# Autodesk Inventor assembly: roka_asemb
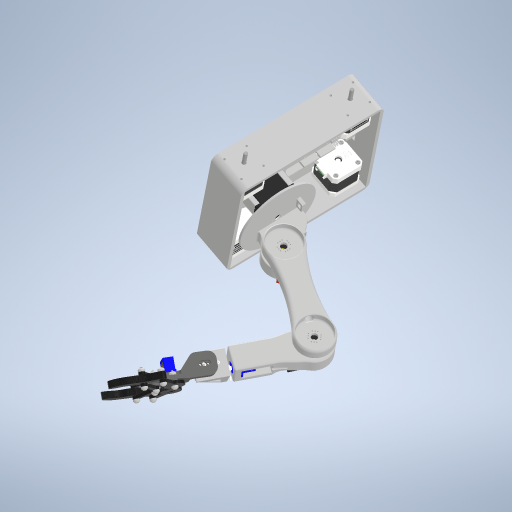
[picture p0: Inventor's stored thumbnail of the model, 512x512]
Saved by Autodesk Inventor 2024 (Build 280153000, 153)
## iProperties
Created: 2023-09-17
Part Number: roka_asemb
Document SubType Name: Assembly
Designer: jebes windows
Author: jebes windows
## Documents named in this file (19)
- C:\Users\jebes windows\Documents\Inventor\Robotska_roka\roka_asemb.iam
- C:\Users\jebes windows\Documents\Inventor\Robotska_roka\vozicek1.ipt
- C:\Users\jebes windows\Documents\Inventor\Robotska_roka\Nema 17 Motor a Pasos 17HS4401\Nema 17 Motor a Pasos 17HS4401.ipt
- C:\Users\jebes windows\Documents\Inventor\Robotska_roka\ArduinoMega_STEP_AP203\ArduinoMega_STEP_AP203.ipt
- C:\Users\jebes windows\Documents\Inventor\Robotska_roka\servo-motor-mg996r-1.snapshot.1(2)\Servo Motor MG996R  With Attachments\Servo Motor MG996R  With Attachments.iam
- C:\Users\jebes windows\Documents\Inventor\Robotska_roka\miza.ipt
- C:\Users\jebes windows\Documents\Inventor\Robotska_roka\pokrow.ipt
- C:\Users\jebes windows\Documents\Inventor\Robotska_roka\roka1.ipt
- C:\Users\jebes windows\Documents\Inventor\Robotska_roka\roka2.ipt
- C:\Users\jebes windows\Documents\Inventor\Robotska_roka\sg90-micro-servo-9g-tower-pro-1.snapshot.3\SG90 - Micro Servo 9g - Tower Pro\SG90 - Micro Servo 9g - Tower Pro.iam
- C:\Users\jebes windows\Documents\Inventor\Robotska_roka\roka3.ipt
- C:\Users\jebes windows\Documents\Inventor\Robotska_roka\Gripper_baza.ipt
- C:\Users\jebes windows\Documents\Inventor\Robotska_roka\Zobnik2.ipt
- C:\Users\jebes windows\Documents\Inventor\Robotska_roka\Zobnik1.ipt
- C:\Users\jebes windows\Documents\Inventor\Robotska_roka\povezava.ipt
- C:\Users\jebes windows\Documents\Inventor\Robotska_roka\Klesce.ipt
- C:\Users\jebes windows\Documents\Inventor\Robotska_roka\sornik1.ipt
- C:\Users\jebes windows\Documents\Inventor\Robotska_roka\matica.ipt
- C:\Users\jebes windows\Documents\Inventor\Robotska_roka\sornik_2.ipt
## Components (43 placed, 18 different names)
1. vozicek1:1 — Rigid:1, Rigid:2, Rigid:3, Rigid:4, Rigid:5, Rigid:6, Rigid:8
2. Nema 17 Motor a Pasos 17HS4401:1 — Rigid:1
3. Nema 17 Motor a Pasos 17HS4401:2 — Rigid:4
4. Nema 17 Motor a Pasos 17HS4401:3 — Rigid:3
5. Nema 17 Motor a Pasos 17HS4401:4 — Rigid:2
6. ArduinoMega_STEP_AP203:1 — Rigid:5
7. Servo Motor MG996R  With Attachments:1 [sub-assembly] — Rigid:6, Rotational:1
8. Servo Motor MG996R  With Attachments:2 [sub-assembly] — Rotational:1, Rigid:7
9. miza:1 — Rigid:7, Rigid:9
10. pokrow:1 — Rigid:8
11. Servo Motor MG996R  With Attachments:3 [sub-assembly] — Rigid:9, Rotational:2
12. Servo Motor MG996R  With Attachments:4 [sub-assembly] — Rotational:2, Rotational:3
13. roka1:1 — Rotational:3, Rotational:5
14. roka2:1 — Rigid:10, Rigid:11
15. Servo Motor MG996R  With Attachments:5 [sub-assembly] — Rigid:10
16. Servo Motor MG996R  With Attachments:6 [sub-assembly] — Rotational:5
17. SG90 - Micro Servo 9g - Tower Pro:1 [sub-assembly] — Rigid:11, Rotational:6
18. SG90 - Micro Servo 9g - Tower Pro:3 [sub-assembly] — Rigid:13, Rotational:9
19. roka3:1 — Rigid:13, Rotational:6
20. SG90 - Micro Servo 9g - Tower Pro:4 [sub-assembly] — Rigid:14, Rotational:10
21. Gripper_baza:1 — Rotational:9, Rigid:14, Rotational:11, Rotational:14, Rotational:15, Rotational:16, Rotational:17, Rotational:29
22. Zobnik2:1 — Rotational:10, Mate:1, Rotational:12, Rotation:1, Rotational:33
23. Zobnik1:1 — Rotational:11, Mate:2, Rotational:13, Rotation:1, Rotational:32, Rotational:34
24. povezava:1 — Rotational:14, Mate:3, Rotational:20, Rotational:24
25. povezava:2 — Rotational:15, Mate:4, Rotational:18, Rotational:22
26. povezava:3 — Mate:6, Rotational:17, Rotational:21, Rotational:25
27. povezava:4 — Mate:5, Rotational:16, Rotational:19, Rotational:23
28. Klesce:1 — Mate:1, Rotational:12, Mate:3, Mate:6, Rotational:31
29. Klesce:2 — Mate:2, Rotational:13, Mate:4, Mate:5, Rotational:27
30. sornik1:1 — Rotational:18
31. matica:1 — Rotational:19
32. sornik1:2 — Rotational:20
33. matica:2 — Rotational:21
34. sornik1:3 — Rotational:22
35. matica:3 — Rotational:23
36. sornik1:4 — Rotational:24
37. matica:4 — Rotational:25
38. matica:5 — Rotational:27
39. matica:6 — Rotational:29
40. matica:7 — Rotational:31
41. sornik_2:1 — Rotational:32
42. sornik_2:2 — Rotational:34
43. sornik_2:3 — Rotational:33
## Relationships (49: RevoluteJoint 29, WeldJoint 13, Mate 6, RelateRotation 1)
- Rigid:1 [WeldJoint]: vozicek1:1 ↔ Nema 17 Motor a Pasos 17HS4401:1
- Rigid:2 [WeldJoint]: vozicek1:1 ↔ Nema 17 Motor a Pasos 17HS4401:4
- Rigid:3 [WeldJoint]: vozicek1:1 ↔ Nema 17 Motor a Pasos 17HS4401:3
- Rigid:4 [WeldJoint]: vozicek1:1 ↔ Nema 17 Motor a Pasos 17HS4401:2
- Rigid:5 [WeldJoint]: vozicek1:1 ↔ ArduinoMega_STEP_AP203:1
- Rigid:6 [WeldJoint]: vozicek1:1 ↔ Servo Motor MG996R  With Attachments:1
- Rotational:1 [RevoluteJoint]: Servo Motor MG996R  With Attachments:1 ↔ Servo Motor MG996R  With Attachments:2
- Rigid:7 [WeldJoint]: Servo Motor MG996R  With Attachments:2 ↔ miza:1
- Rigid:8 [WeldJoint]: vozicek1:1 ↔ pokrow:1
- Rigid:9 [WeldJoint]: miza:1 ↔ Servo Motor MG996R  With Attachments:3
- Rotational:2 [RevoluteJoint]: Servo Motor MG996R  With Attachments:3 ↔ Servo Motor MG996R  With Attachments:4
- Rotational:3 [RevoluteJoint]: Servo Motor MG996R  With Attachments:4 ↔ roka1:1
- [RevoluteJoint]: Servo Motor MG996R  With Attachments:5 ↔ Servo Motor MG996R  With Attachments:6
- Rigid:10 [WeldJoint]: roka2:1 ↔ Servo Motor MG996R  With Attachments:5
- Rotational:5 [RevoluteJoint]: roka1:1 ↔ Servo Motor MG996R  With Attachments:6
- Rigid:11 [WeldJoint]: roka2:1 ↔ SG90 - Micro Servo 9g - Tower Pro:1
- Rigid:13 [WeldJoint]: SG90 - Micro Servo 9g - Tower Pro:3 ↔ roka3:1
- Rotational:6 [RevoluteJoint]: SG90 - Micro Servo 9g - Tower Pro:1 ↔ roka3:1
- Rotational:9 [RevoluteJoint]: SG90 - Micro Servo 9g - Tower Pro:3 ↔ Gripper_baza:1
- Rigid:14 [WeldJoint]: SG90 - Micro Servo 9g - Tower Pro:4 ↔ Gripper_baza:1
- Rotational:10 [RevoluteJoint]: SG90 - Micro Servo 9g - Tower Pro:4 ↔ Zobnik2:1
- Rotational:11 [RevoluteJoint]: Gripper_baza:1 ↔ Zobnik1:1
- Mate:1: Zobnik2:1 ↔ Klesce:1
- Rotational:12 [RevoluteJoint]: Zobnik2:1 ↔ Klesce:1
- Mate:2: Zobnik1:1 ↔ Klesce:2
- Rotational:13 [RevoluteJoint]: Zobnik1:1 ↔ Klesce:2
- Rotational:14 [RevoluteJoint]: Gripper_baza:1 ↔ povezava:1
- Mate:3: povezava:1 ↔ Klesce:1
- Rotational:15 [RevoluteJoint]: Gripper_baza:1 ↔ povezava:2
- Mate:4: povezava:2 ↔ Klesce:2
- Mate:5: povezava:4 ↔ Klesce:2
- Mate:6: povezava:3 ↔ Klesce:1
- Rotational:16 [RevoluteJoint]: Gripper_baza:1 ↔ povezava:4
- Rotational:17 [RevoluteJoint]: Gripper_baza:1 ↔ povezava:3
- Rotation:1 [RelateRotation] (1 ul): Zobnik2:1 ↔ Zobnik1:1
- Rotational:18 [RevoluteJoint]: povezava:2 ↔ sornik1:1
- Rotational:19 [RevoluteJoint]: povezava:4 ↔ matica:1
- Rotational:20 [RevoluteJoint]: povezava:1 ↔ sornik1:2
- Rotational:21 [RevoluteJoint]: povezava:3 ↔ matica:2
- Rotational:22 [RevoluteJoint]: povezava:2 ↔ sornik1:3
- Rotational:23 [RevoluteJoint]: povezava:4 ↔ matica:3
- Rotational:24 [RevoluteJoint]: povezava:1 ↔ sornik1:4
- Rotational:25 [RevoluteJoint]: povezava:3 ↔ matica:4
- Rotational:27 [RevoluteJoint]: Klesce:2 ↔ matica:5
- Rotational:29 [RevoluteJoint]: Gripper_baza:1 ↔ matica:6
- Rotational:31 [RevoluteJoint]: Klesce:1 ↔ matica:7
- Rotational:32 [RevoluteJoint]: Zobnik1:1 ↔ sornik_2:1
- Rotational:33 [RevoluteJoint]: Zobnik2:1 ↔ sornik_2:3
- Rotational:34 [RevoluteJoint]: Zobnik1:1 ↔ sornik_2:2
## Named parameters: d15_d11 = 0 mm, d16_d12 = -36.858233 deg
